# Autodesk Inventor assembly: TheCarrier&Jig
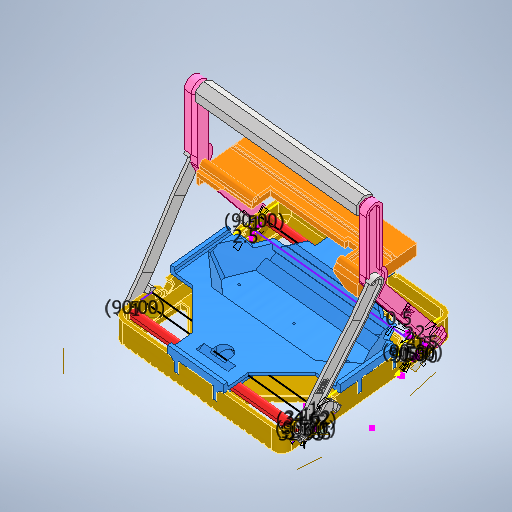
[picture p0: Inventor's stored thumbnail of the model, 512x512]
Saved by Autodesk Inventor 2025.1 (Build 291241000, 241)
## iProperties
Created: 2026-05-10
Part Number: TheCarrier&Jig
Document SubType Name: Assembly
Designer: User
Author: User
## Documents named in this file (11)
- D:\One Drive\OneDrive - Politeknik Sultan Salahuddin Abdul Aziz Shah\Documents\Inventor\RobosotPSA\TheCarrier&Jig.iam
- D:\One Drive\OneDrive - Politeknik Sultan Salahuddin Abdul Aziz Shah\Documents\Inventor\RobosotPSA\RobotStand.ipt
- D:\One Drive\OneDrive - Politeknik Sultan Salahuddin Abdul Aziz Shah\Documents\Inventor\RobosotPSA\RobotStandBase.ipt
- D:\One Drive\OneDrive - Politeknik Sultan Salahuddin Abdul Aziz Shah\Documents\Inventor\RobosotPSA\RobotStandHandle.ipt
- D:\One Drive\OneDrive - Politeknik Sultan Salahuddin Abdul Aziz Shah\Documents\Inventor\RobosotPSA\TheHandle_Left.ipt
- D:\One Drive\OneDrive - Politeknik Sultan Salahuddin Abdul Aziz Shah\Documents\Inventor\RobosotPSA\TheHandle_Right.ipt
- D:\One Drive\OneDrive - Politeknik Sultan Salahuddin Abdul Aziz Shah\Documents\Inventor\RobosotPSA\TheHandle_LeftBack.ipt
- D:\One Drive\OneDrive - Politeknik Sultan Salahuddin Abdul Aziz Shah\Documents\Inventor\RobosotPSA\TheHandle_RightBack.ipt
- D:\One Drive\OneDrive - Politeknik Sultan Salahuddin Abdul Aziz Shah\Documents\Inventor\RobosotPSA\BaseShaft.ipt
- D:\One Drive\OneDrive - Politeknik Sultan Salahuddin Abdul Aziz Shah\Documents\Inventor\RobosotPSA\TheHandleBar.ipt
- D:\One Drive\OneDrive - Politeknik Sultan Salahuddin Abdul Aziz Shah\Documents\Inventor\RobosotPSA\Lock1.ipt
## Components (14 placed, 10 different names)
1. RobotStand:1 — Mate:1, Flush:1, Flush:2
2. RobotStandBase:1 — Mate:1, Flush:1, Flush:2, Flush:3, Flush:5, Mate:2, Mate:3, Mate:5, Mate:6, Flush:6, Flush:7, Mate:8, Mate:11, Mate:12, Mate:13, Mate:16, Mate:17, Flush:9, Mate:18
3. RobotStandHandle:1 — Flush:3, Flush:5, Mate:4, Mate:7
4. TheHandle_Left:1 — Mate:2, Mate:3, Mate:4
5. TheHandle_Right:1 — Mate:5, Mate:6, Mate:7, Flush:8
6. TheHandle_LeftBack:1 — Flush:6
7. TheHandle_RightBack:1 — Flush:7
8. BaseShaft:1
9. BaseShaft:2
10. TheHandleBar:1 — Flush:8
11. Lock1:1
12. Lock1:2 — Mate:8, Mate:11, Mate:12, Mate:13
13. Lock1:3 — Mate:18
14. Lock1:4 — Mate:16, Mate:17, Flush:9
## Relationships (22: Mate 14, Flush 8)
- Mate:1: RobotStand:1 ↔ RobotStandBase:1
- Flush:1: RobotStand:1 ↔ RobotStandBase:1
- Flush:2: RobotStand:1 ↔ RobotStandBase:1
- Flush:3 (46.8 mm): RobotStandBase:1 ↔ RobotStandHandle:1
- Flush:5 (6.146 mm): RobotStandBase:1 ↔ RobotStandHandle:1
- Mate:2: RobotStandBase:1 ↔ TheHandle_Left:1
- Mate:3: RobotStandBase:1 ↔ TheHandle_Left:1
- Mate:4: RobotStandHandle:1 ↔ TheHandle_Left:1
- Mate:5: RobotStandBase:1 ↔ TheHandle_Right:1
- Mate:6: RobotStandBase:1 ↔ TheHandle_Right:1
- Mate:7: RobotStandHandle:1 ↔ TheHandle_Right:1
- Flush:6: RobotStandBase:1 ↔ TheHandle_LeftBack:1
- Flush:7: RobotStandBase:1 ↔ TheHandle_RightBack:1
- Flush:8: TheHandle_Right:1 ↔ TheHandleBar:1
- Mate:8: RobotStandBase:1 ↔ Lock1:2
- Mate:11: RobotStandBase:1 ↔ Lock1:2
- Mate:12: RobotStandBase:1 ↔ Lock1:2
- Mate:13: RobotStandBase:1 ↔ Lock1:2
- Mate:16: RobotStandBase:1 ↔ Lock1:4
- Mate:17: RobotStandBase:1 ↔ Lock1:4
- Flush:9: RobotStandBase:1 ↔ Lock1:4
- Mate:18: RobotStandBase:1 ↔ Lock1:3
